# Autodesk Inventor assembly: Finished
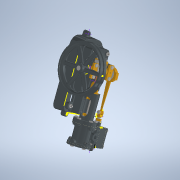
[picture p0: Inventor's stored thumbnail of the model, 180x180]
Saved by Autodesk Inventor 2020 (Build 240168000, 168)
## iProperties
Created: 2021-10-28
Part Number: Finished
Document SubType Name: Assembly
Designer: simon.erikssonwestl
Author: simon.erikssonwestl
## Documents named in this file (16)
- C:\Users\simon.erikssonwestl\Documents\Inventor\Ång\Assemblies\Finished.iam
- C:\Users\simon.erikssonwestl\Documents\Inventor\Ång\Assemblies\Cylinder.iam
- C:\Users\simon.erikssonwestl\Documents\Inventor\Ång\Assemblies\Slider.iam
- C:\Users\simon.erikssonwestl\Documents\Inventor\Content Center Files\R2020\en-US\BS 4464 A\BS 4464 - M6 Form A.ipt
- C:\Users\simon.erikssonwestl\Documents\Inventor\Ång\Part25.ipt
- C:\Users\simon.erikssonwestl\Documents\Inventor\Ång\Assemblies\Exentric strap.iam
- C:\Users\simon.erikssonwestl\Documents\Inventor\Content Center Files\R2020\en-US\AS 1110\AS 1110 - M2,5 x 10.ipt
- C:\Users\simon.erikssonwestl\Documents\Inventor\Content Center Files\R2020\en-US\AS 1112 (2)\AS 1112 - M2,5  Type 5.ipt
- C:\Users\simon.erikssonwestl\Documents\Inventor\Ång\Assemblies\Crank.iam
- C:\Users\simon.erikssonwestl\Documents\Inventor\Ång\Part11.ipt
- C:\Users\simon.erikssonwestl\Documents\Inventor\Content Center Files\R2020\en-US\AS 1110\AS 1110 - M2,5 x 8.ipt
- C:\Users\simon.erikssonwestl\Documents\Inventor\Ång\Assemblies\Piston.iam
- C:\Users\simon.erikssonwestl\Documents\Inventor\Ång\Assemblies\Connection rod.iam
- C:\Users\simon.erikssonwestl\Documents\Inventor\Ång\Part32.ipt
- C:\Users\simon.erikssonwestl\Documents\Inventor\Ång\Part31.ipt
- C:\Users\simon.erikssonwestl\Documents\Inventor\Content Center Files\R2020\en-US\BS 4464 A\BS 4464 - M8 Form A.ipt
## Components (19 placed, 15 different names)
1. Cylinder:1 [sub-assembly] — Mate:3, Mate:12, Mate:15, Mate:17, Mate:26, Mate:27, Angle:1, Mate:39, Mate:40, Mate:41
2. BS 4464 Form A M6 Form A:1 — Mate:3, Mate:5, Mate:28
3. Part25:1 — Mate:5, Mate:29
4. Exentric strap:1 [sub-assembly] — Mate:13, Flush:1, Mate:30, Mate:34
5. AS 1110 - Metric M2,5 x 10:1 — Mate:10, Mate:31, Mate:32
6. AS 1112 (2) - Metric M2,5  Type 5:1 — Mate:10, Mate:33
7. Crank:1 [sub-assembly] — Mate:12, Mate:13, Flush:1, Mate:14, Mate:16, Mate:35, Spin
8. Part11:1 — Mate:14, Mate:15, Mate:18, Mate:19, Mate:24, Mate:25, Spin
9. Part11:2 — Mate:16, Mate:17, Mate:20, Mate:21, Mate:22, Mate:23
10. AS 1110 - Metric M2,5 x 8:1 — Mate:18, Mate:24
11. AS 1110 - Metric M2,5 x 8:2 — Mate:19, Mate:25
12. AS 1110 - Metric M2,5 x 8:3 — Mate:20, Mate:22
13. AS 1110 - Metric M2,5 x 8:4 — Mate:21, Mate:23
14. Piston:1 [sub-assembly] — Mate:26, Mate:36, Mate:38
15. Slider:1 [sub-assembly] — Mate:27, Angle:1, Mate:28, Mate:29, Mate:30, Mate:31, Mate:32, Mate:33, Mate:34
16. Connection rod:1 [sub-assembly] — Mate:35, Mate:36, Mate:37, Flush:2, Mate:38
17. Part32:1 — Mate:37, Flush:2
18. Part31:1 — Mate:39, Mate:42
19. BS 4464 Form A M8 Form A:1 — Mate:40, Mate:41, Mate:42
## Relationships (38: Mate 34, Flush 2, Angle 2)
- Mate:3: Cylinder:1 ↔ BS 4464 Form A M6 Form A:1
- Mate:5: BS 4464 Form A M6 Form A:1 ↔ Part25:1
- Mate:10: AS 1110 - Metric M2,5 x 10:1 ↔ AS 1112 (2) - Metric M2,5  Type 5:1
- Mate:12: Cylinder:1 ↔ Crank:1
- Mate:13: Exentric strap:1 ↔ Crank:1
- Flush:1: Exentric strap:1 ↔ Crank:1
- Mate:14: Crank:1 ↔ Part11:1
- Mate:15: Cylinder:1 ↔ Part11:1
- Mate:16: Crank:1 ↔ Part11:2
- Mate:17: Cylinder:1 ↔ Part11:2
- Mate:18: Part11:1 ↔ AS 1110 - Metric M2,5 x 8:1
- Mate:19: Part11:1 ↔ AS 1110 - Metric M2,5 x 8:2
- Mate:20: Part11:2 ↔ AS 1110 - Metric M2,5 x 8:3
- Mate:21: Part11:2 ↔ AS 1110 - Metric M2,5 x 8:4
- Mate:22: Part11:2 ↔ AS 1110 - Metric M2,5 x 8:3
- Mate:23: Part11:2 ↔ AS 1110 - Metric M2,5 x 8:4
- Mate:24: Part11:1 ↔ AS 1110 - Metric M2,5 x 8:1
- Mate:25: Part11:1 ↔ AS 1110 - Metric M2,5 x 8:2
- Mate:26: Cylinder:1 ↔ Piston:1
- Mate:27: Cylinder:1 ↔ Slider:1
- Angle:1 (180 deg): Cylinder:1 ↔ Slider:1
- Mate:28: BS 4464 Form A M6 Form A:1 ↔ Slider:1
- Mate:29: Part25:1 ↔ Slider:1
- Mate:30: Exentric strap:1 ↔ Slider:1
- Mate:31: AS 1110 - Metric M2,5 x 10:1 ↔ Slider:1
- Mate:32: AS 1110 - Metric M2,5 x 10:1 ↔ Slider:1
- Mate:33: AS 1112 (2) - Metric M2,5  Type 5:1 ↔ Slider:1
- Mate:34 (0.5 mm): Exentric strap:1 ↔ Slider:1
- Mate:35: Crank:1 ↔ Connection rod:1
- Mate:36: Piston:1 ↔ Connection rod:1
- Mate:37: Connection rod:1 ↔ Part32:1
- Flush:2: Connection rod:1 ↔ Part32:1
- Mate:38 (0.5 mm): Piston:1 ↔ Connection rod:1
- Mate:39: Cylinder:1 ↔ Part31:1
- Mate:40: Cylinder:1 ↔ BS 4464 Form A M8 Form A:1
- Mate:41: Cylinder:1 ↔ BS 4464 Form A M8 Form A:1
- Mate:42: Part31:1 ↔ BS 4464 Form A M8 Form A:1
- Spin [Angle] (0 deg): Crank:1 ↔ Part11:1
